# Autodesk Inventor assembly: CDJ2B16-15Z-B(0_1_0)
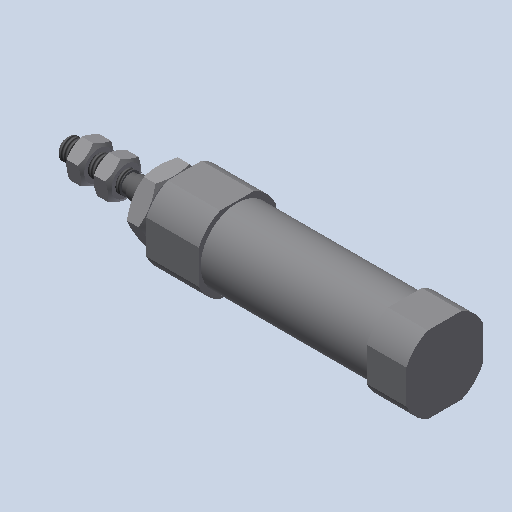
[picture p0: Inventor's stored thumbnail of the model, 512x512]
Saved by Autodesk Inventor 2025.1 (Build 291241000, 241)
## iProperties
Category: PARTsolutions
Company: SMC
Created: 2024-03-16
Part Number: CDJ2B16-15Z-B(0_1_0)
Catalog Web Link: www.cadenas.de
Description: CJ2-Z/CDJ2-Z-Air Cylinder/Standard: Double Acting Single Rod
Vendor: SMC
Document SubType Name: Assembly
Designer: psAdmin
Manufacturer: SMC
Mass: 14.8803 g
Surface Area: 87.7268 cm^2
Volume: 14.8803 cm^3
PSOL_IDENT_0: {$CADENAS_DATA/23d-libs/smc_jp/actuator/standard_air_cylinder/cj2/cj2_z_asmtab.prj},313 {VTYP=3D},{S
PSOL_IDENT_1: TYP=ASSTAB},{NB=CDJ2B16-15Z-B(0_1_0)},{LINA=CDJ2B16-15Z-B},{NN=CJ2-Z/CDJ2-Z},{DATE=01.03.2024 06:19:
PSOL_IDENT_2: 42},{GEOMDATE=25.05.2023 02:41:22},{VERSION=},{LINEID=410},{WBVAR=MAGNET,AUTOSWITCH,LEAD,NUMBER,CUSH
PSOL_IDENT_3: ION,STROKE,POS,PORT,STOP,BRACKET,RODB,MOUNTING,OMSC,OMSCXC3,OMSCXC51,THREAD},{WBNUMERIC=STROKE,POS}
PSOL_IDENT_4: {NB=CDJ2B16-15Z-B(0_1_0)},{LINA=CDJ2B16-15Z-B},{KT=DUMMY},{NENN=CDJ2B16-15Z},{ORDER=CDJ2B16-15Z-B},
PSOL_IDENT_5: {BORE=16},{MOUNT=(B) Basic},{MOUNTX=B},{MAGNET=D},{AUTOSWITCH=},{AUTOSWX= '','(-) Without autoswitch'
PSOL_IDENT_6: ,'-M9N','M9N','-M9P','M9P','-M9B','M9B','-H7C','H7C','-M9NW','M9NW','-M9PW','M9PW','-M9BW','M9BW','-
PSOL_IDENT_7: M9NA','M9NA','-M9PA','M9PA','-M9BA','M9BA','-H7NF','H7NF','-A96','A96','-A93','A93','-A90','A90','-C
PSOL_IDENT_8: 73C','C73C','-C80C','C80C','-M9NV','M9NV','-M9PV','M9PV','-M9BV','M9BV','-M9NWV','M9NWV','-M9PWV','M
PSOL_IDENT_9: 9PWV','-M9BWV','M9BWV','-M9NAV','M9NAV','-M9PAV','M9PAV','-M9BAV','M9BAV','-A96V','A96V','-A93V','A9
PSOL_IDENT_10: 3V','-A90V','A90V','-J79C','J79C','-F79F','F79F','-A72','A72','-A72H','A72H','-A73C','A73C','-A80C','
PSOL_IDENT_11: A80C','-A79W','A79W' },{LEAD=},{LEADX= '','N/A' },{NUMBER=},{CUSHION=},{CUSHIONX= '','(-) Rubber cus
PSOL_IDENT_12: hion','A','(A) Air cushion' },{SWSIGNX= '','N/A' },{STROKE=15},{STDSTROKE=15,30,45,60,75,100,125,150
PSOL_IDENT_13: ,175,200},{STROKE1X=[5:400/1]},{SMIN=5},{SMINASW1=10},{SMINASW2=15},{SMAX1=400},{POS=0},{PORT=},{STO
PSOL_IDENT_14: P=1},{COM=Please confirm the conditions of use with SMC},{COM1=-},{BRACKET=},{RODB=},{RODBX= '', '(-
PSOL_IDENT_15: ) None', 'V', '(V) Single knuckle joint', 'W'  , '(W) Double knuckle joint', 'T', '(T) Rod end cap (
PSOL_IDENT_16: Flat type)', 'U'  , '(U) Rod end cap (Round type)' },{MOUNTING=-B},{OMSC=},{OMSCXC3=},{OMSCXC51=},{T
PSOL_IDENT_17: HREAD=0},{MOUNTINGX='-A','(A) Rail mounting','-B','(B) Band mounting'},{BRACKETX='','N/A'},{PORTX=''
PSOL_IDENT_18: , '(-) Perpendicular to axis', 'R', '(R) Axial'},{SW=B},{OMSCX= '','(-) None','-XB9','(XB9) Low spee
PSOL_IDENT_19: d cylinder (10 to 50 mm/s)','-XC22','(XC22) Fluororubber seals','-XC85','(XC85) Grease specification
PSOL_IDENT_20: for food processing machines', '-X446'  , '(X446) PTFE grease' },{A=2.5},{XC3= '','(-) None','-XC3A
PSOL_IDENT_21: B','(XC3AB) Rod port location viewed: A,Head port location viewed: B','-XC3AC','(XC3AC) Rod port loc
PSOL_IDENT_22: ation viewed: A,Head port location viewed: C','-XC3AD','(XC3AD) Rod port location viewed: A,Head por
PSOL_IDENT_23: t location viewed: D','-XC3BA','(XC3BA) Rod port location viewed: B,Head port location viewed: A','-
PSOL_IDENT_24: XC3BB','(XC3BB) Rod port location viewed: B,Head port location viewed: B','-XC3BC','(XC3BC) Rod port
PSOL_IDENT_25: location viewed: B,Head port location viewed: C','-XC3BD','(XC3BD) Rod port location viewed: B,Head
PSOL_IDENT_26: port location viewed: D','-XC3CA','(XC3CA) Rod port location viewed: C,Head port location viewed: A'
PSOL_IDENT_27: ,'-XC3CB','(XC3CB) Rod port location viewed: C,Head port location viewed: B','-XC3CC','(XC3CC) Rod p
PSOL_IDENT_28: ort location viewed: C,Head port location viewed: C','-XC3CD','(XC3CD) Rod port location viewed: C,H
PSOL_IDENT_29: ead port location viewed: D','-XC3DA','(XC3DA) Rod port location viewed: D,Head port location viewed
PSOL_IDENT_30: : A','-XC3DB','(XC3DB) Rod port location viewed: D,Head port location viewed: B','-XC3DC','(XC3DC) R
PSOL_IDENT_31: od port location viewed: D,Head port location viewed: C','-XC3DD','(XC3DD) Rod port location viewed:
PSOL_IDENT_32: D,Head port location viewed: D' },{XC51= '','(-) None','-XC51H4','(XC51H4) Hose nipple type: ø4/2.5
PSOL_IDENT_33: with restriction','-XC51H6','(XC51H6) Hose nipple type: ø6/4 with restriction','-XC51MH4','(XC51MH4
PSOL_IDENT_34: ) Hose nipple type: ø4/2.5 without restriction','-XC51MH6','(XC51MH6) Hose nipple type: ø6/4 without
PSOL_IDENT_35: restriction' },{BMP=B},{PPATH=cj2_z/assembly/cj2_z_asmsbl.prj},{OMSCXX= '','(-) None','-XB9','(XB9)
PSOL_IDENT_36: Low speed cylinder (10 to 50 mm/s)','-XC22','(XC22) Fluororubber seals','-XC85','(XC85) Grease spec
PSOL_IDENT_37: ification for food processing machines', '-X446' , '(X446) PTFE grease' }
NB: CDJ2B16-15Z-B(0_1_0)
NN: CJ2-Z/CDJ2-Z
NT: Air Cylinder/Standard: Double Acting Single Rod
NBSYN: $ORDER.($POS._$STOP._$THREAD.)
LINA: CDJ2B16-15Z-B
CATALOG: SMC (JP
BORE: 16
MOUNT: (B) Basic
MAGNET: (D) With magnet
AUTOSWITCH: (-) Without autoswitch
LEAD: N/A
NUMBER: N/A
CUSHION: (-) Rubber cushion
STROKE: 15
POS: 0
PORT: (-) Perpendicular to axis
STOP: Manufacturable stroke
COM: Please confirm the conditions of use with SMC
COM1: -
BRACKET: N/A
RODB: (-) None
MOUNTING: (B) Band mounting
OMSC: (-) None
OMSCXC3: (-) None
OMSCXC51: (-) None
THREAD: on
SUPPLIER: SMC
ARTICLENO: CDJ2B16-15Z-B(0_1_0)
BOMINFO: CDJ2B16-15Z-B
CREATOR: CADENAS GmbH
Title: CDJ2B16-15Z-B
Author: Cadenas PARTsolutions
Comments: Air Cylinder/Standard: Double Acting Single Rod
## Documents named in this file (5)
- C:\Users\haruy\Documents\ロボコン\NHK2025\cad\000_parts\エアシリンダー\airclinder\CDJ2B16-15Z-B(0_1_0).iam
- C:\Users\haruy\Documents\ロボコン\NHK2025\cad\000_parts\エアシリンダー\airclinder\CJ2B16-15Z-B(1_0)_BODY.ipt
- C:\Users\haruy\Documents\ロボコン\NHK2025\cad\000_parts\エアシリンダー\airclinder\CJ2B16-15Z_ROD.ipt
- C:\Users\haruy\Documents\ロボコン\NHK2025\cad\000_parts\エアシリンダー\airclinder\NTJ-015C.ipt
- C:\Users\haruy\Documents\ロボコン\NHK2025\cad\000_parts\エアシリンダー\airclinder\SNJ-016C.ipt
## Components (5 placed, 4 different names)
1. CJ2B16-15Z-B(1_0)_BODY:1 — body_XY@1 <-> ROD_BODY_XY@2, body_Z@1 <-> ROD_BODY_Z@2, body_XY@1 <-> ntj_XY@5, body_Z@1 <-> ntj_Z@5, body_YZ@1 <-> ntj_YZ@5
2. CJ2B16-15Z_ROD:1 — body_XY@1 <-> ROD_BODY_XY@2, body_Z@1 <-> ROD_BODY_Z@2, rodnt1_XY@2 <-> ntj_XY@3, rodnt1_Z@2 <-> ntj_Z@3, rodnt1_YZ@2 <-> ntj_YZ@3, rodnt1_XY@2 <-> ntj_XY@4, rodnt1_Z@2 <-> ntj_Z@4, rodnt1_YZ@2 <-> ntj_YZ@4
3. NTJ-015C:1 — rodnt1_XY@2 <-> ntj_XY@3, rodnt1_Z@2 <-> ntj_Z@3, rodnt1_YZ@2 <-> ntj_YZ@3
4. NTJ-015C:2 — rodnt1_XY@2 <-> ntj_XY@4, rodnt1_Z@2 <-> ntj_Z@4, rodnt1_YZ@2 <-> ntj_YZ@4
5. SNJ-016C:1 — body_XY@1 <-> ntj_XY@5, body_Z@1 <-> ntj_Z@5, body_YZ@1 <-> ntj_YZ@5
## Relationships (11: Mate 7, Angle 3, Flush 1)
- body_XY@1 <-> ROD_BODY_XY@2 [Mate]: CJ2B16-15Z-B(1_0)_BODY:1 ↔ CJ2B16-15Z_ROD:1
- body_Z@1 <-> ROD_BODY_Z@2 [Mate]: CJ2B16-15Z-B(1_0)_BODY:1 ↔ CJ2B16-15Z_ROD:1
- rodnt1_XY@2 <-> ntj_XY@3 [Mate] (2.5 mm): CJ2B16-15Z_ROD:1 ↔ NTJ-015C:1
- rodnt1_Z@2 <-> ntj_Z@3 [Mate]: CJ2B16-15Z_ROD:1 ↔ NTJ-015C:1
- rodnt1_YZ@2 <-> ntj_YZ@3 [Angle] (0 deg): CJ2B16-15Z_ROD:1 ↔ NTJ-015C:1
- rodnt1_XY@2 <-> ntj_XY@4 [Flush]: CJ2B16-15Z_ROD:1 ↔ NTJ-015C:2
- rodnt1_Z@2 <-> ntj_Z@4 [Mate]: CJ2B16-15Z_ROD:1 ↔ NTJ-015C:2
- rodnt1_YZ@2 <-> ntj_YZ@4 [Angle] (0 deg): CJ2B16-15Z_ROD:1 ↔ NTJ-015C:2
- body_XY@1 <-> ntj_XY@5 [Mate] (2.3 mm): CJ2B16-15Z-B(1_0)_BODY:1 ↔ SNJ-016C:1
- body_Z@1 <-> ntj_Z@5 [Mate]: CJ2B16-15Z-B(1_0)_BODY:1 ↔ SNJ-016C:1
- body_YZ@1 <-> ntj_YZ@5 [Angle] (0 deg): CJ2B16-15Z-B(1_0)_BODY:1 ↔ SNJ-016C:1
